# Autodesk Inventor assembly: 5x22BoltWasher
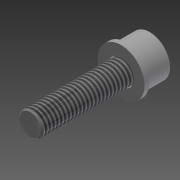
[picture p0: Inventor's stored thumbnail of the model, 180x180]
Saved by Autodesk Inventor 2015 (Build 190159000, 159)
## iProperties
Created: 2014-02-08
Part Number: 5x22BoltWasher
Document SubType Name: Assembly
Designer: Jack
Author: Jack
## Documents named in this file (3)
- C:\Users\Jack\Sync\MendelMax1.5\InventorParts\Hardware\BoltWashers\5x22BoltWasher.iam
- C:\Users\Jack\Sync\MendelMax1.5\InventorParts\Hardware\Bolts\M5x22SHCS.ipt
- C:\Users\Jack\Sync\MendelMax1.5\InventorParts\Hardware\Washers\M5Washer.ipt
## Components (2 placed, 2 different names)
1. M5x22SHCS:1 — Mate:1, Mate:2
2. M5Washer:1 — Mate:1, Mate:2
## Relationships (2: Mate 2)
- Mate:1: M5x22SHCS:1 ↔ M5Washer:1
- Mate:2: M5x22SHCS:1 ↔ M5Washer:1
